# Autodesk Inventor assembly: 6_7_2022_Assembly1
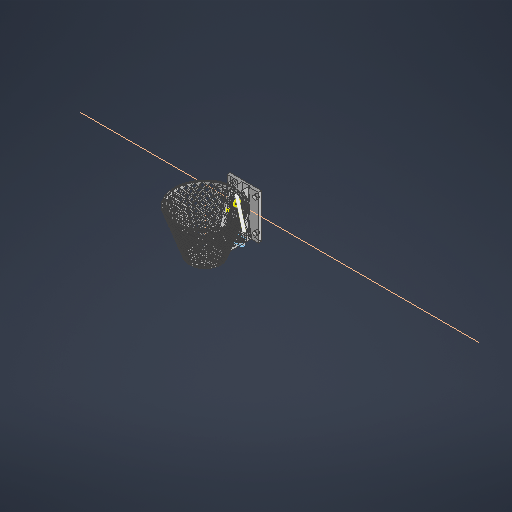
[picture p0: Inventor's stored thumbnail of the model, 512x512]
Saved by Autodesk Inventor 2025 (Build 290162000, 162)
## iProperties
Created: 2022-06-07
Part Number: 6_7_2022_Assembly1
Document SubType Name: Assembly
Designer: micha
Author: micha
## Documents named in this file (8)
- C:\Users\Admin\Desktop\rat basketball\rat_basketball\Hoop assembly\hoop assembly.iam
- C:\Users\Admin\Desktop\rat basketball\rat_basketball\Hoop assembly\HOOP.ipt
- C:\Users\Admin\Desktop\rat basketball\rat_basketball\Hoop assembly\IR sensorIR Optical Sensor Module.ipt
- C:\Users\Admin\Desktop\rat basketball\rat_basketball\Hoop assembly\sensor arm v3.ipt
- C:\Users\Admin\Desktop\rat basketball\rat_basketball\Hoop assembly\684AZZ.iam
- C:\Users\Admin\Desktop\rat basketball\rat_basketball\Hoop assembly\DIN EN ISO 4762 - M4 x 25.ipt
- C:\Users\Admin\Desktop\rat basketball\rat_basketball\Hoop assembly\ISO 7089 - 4 - 140 HV(1).ipt
- C:\Users\Admin\Desktop\rat basketball\rat_basketball\Hoop assembly\ISO 4032 - M4 - ISO.ipt
## Components (8 placed, 7 different names)
1. HOOP:1 — Mate:1, Flush:1, Flush:2, Mate:2, Mate:3, Mate:4, Mate:5, Mate:6, Mate:7, Mate:8, Mate:10
2. IR sensorIR Optical Sensor Module:1 — Mate:1, Flush:1
3. sensor arm v3:1 — Flush:2, Flush:3, Mate:9, Mate:10
4. 684AZZ:1 [sub-assembly] — Mate:9
5. 684AZZ:2 [sub-assembly] — Flush:3
6. DIN EN ISO 4762 M4 x 25:1 — Mate:5, Mate:6
7. ISO 7089 4:1 — Mate:7, Mate:8, Insert:1
8. ISO 4032 M4:1 — Insert:1
## Relationships (14: Mate 10, Flush 3, Insert 1)
- Mate:1: HOOP:1 ↔ IR sensorIR Optical Sensor Module:1
- Flush:1: HOOP:1 ↔ IR sensorIR Optical Sensor Module:1
- Flush:2: HOOP:1 ↔ sensor arm v3:1
- Flush:3: sensor arm v3:1 ↔ 684AZZ:2
- Mate:2: HOOP:1
- Mate:3: HOOP:1
- Mate:4: HOOP:1
- Mate:5: HOOP:1 ↔ DIN EN ISO 4762 M4 x 25:1
- Mate:6: HOOP:1 ↔ DIN EN ISO 4762 M4 x 25:1
- Mate:7: HOOP:1 ↔ ISO 7089 4:1
- Mate:8: HOOP:1 ↔ ISO 7089 4:1
- Insert:1: ISO 7089 4:1 ↔ ISO 4032 M4:1
- Mate:9: sensor arm v3:1 ↔ 684AZZ:1
- Mate:10: HOOP:1 ↔ sensor arm v3:1
